# Autodesk Inventor assembly: Shield_100
(part 2 of 2)
- C:\Users\dvorakj\Documents\Inventor\Bakalarka\altium export\NUCLEO-F411RE_PCB_TOP_Designators_Varsay_X_8Dlan_416.ipt
- C:\Users\dvorakj\Documents\Inventor\Bakalarka\altium export\NUCLEO-F411RE_PCB_TOP_Designators_Varsay_X_8Dlan_417.ipt
- C:\Users\dvorakj\Documents\Inventor\Bakalarka\altium export\NUCLEO-F411RE_PCB_TOP_Designators_Varsay_X_8Dlan_418.ipt
- C:\Users\dvorakj\Documents\Inventor\Bakalarka\altium export\NUCLEO-F411RE_PCB_TOP_Designators_Varsay_X_8Dlan_419.ipt
- C:\Users\dvorakj\Documents\Inventor\Bakalarka\altium export\NUCLEO-F411RE_PCB_TOP_Designators_Varsay_X_8Dlan_420.ipt
- C:\Users\dvorakj\Documents\Inventor\Bakalarka\altium export\NUCLEO-F411RE_PCB_TOP_Designators_Varsay_X_8Dlan_421.ipt
- C:\Users\dvorakj\Documents\Inventor\Bakalarka\altium export\NUCLEO-F411RE_PCB_TOP_Designators_Varsay_X_8Dlan_422.ipt
- C:\Users\dvorakj\Documents\Inventor\Bakalarka\altium export\NUCLEO-F411RE_PCB_TOP_Designators_Varsay_X_8Dlan_423.ipt
- C:\Users\dvorakj\Documents\Inventor\Bakalarka\altium export\NUCLEO-F411RE_PCB_TOP_Designators_Varsay_X_8Dlan_424.ipt
- C:\Users\dvorakj\Documents\Inventor\Bakalarka\altium export\NUCLEO-F411RE_PCB_TOP_Designators_Varsay_X_8Dlan_425.ipt
- C:\Users\dvorakj\Documents\Inventor\Bakalarka\altium export\NUCLEO-F411RE_PCB_TOP_Designators_Varsay_X_8Dlan_426.ipt
- C:\Users\dvorakj\Documents\Inventor\Bakalarka\altium export\NUCLEO-F411RE_PCB_TOP_Designators_Varsay_X_8Dlan_427.ipt
- C:\Users\dvorakj\Documents\Inventor\Bakalarka\altium export\NUCLEO-F411RE_PCB_TOP_Designators_Varsay_X_8Dlan_428.ipt
- C:\Users\dvorakj\Documents\Inventor\Bakalarka\altium export\NUCLEO-F411RE_PCB_TOP_Designators_Varsay_X_8Dlan_429.ipt
- C:\Users\dvorakj\Documents\Inventor\Bakalarka\altium export\NUCLEO-F411RE_PCB_TOP_Designators_Varsay_X_8Dlan_430.ipt
- C:\Users\dvorakj\Documents\Inventor\Bakalarka\altium export\NUCLEO-F411RE_PCB_TOP_Designators_Varsay_X_8Dlan_431.ipt
- C:\Users\dvorakj\Documents\Inventor\Bakalarka\altium export\NUCLEO-F411RE_PCB_TOP_Designators_Varsay_X_8Dlan_432.ipt
- C:\Users\dvorakj\Documents\Inventor\Bakalarka\altium export\NUCLEO-F411RE_PCB_TOP_Designators_Varsay_X_8Dlan_433.ipt
- C:\Users\dvorakj\Documents\Inventor\Bakalarka\altium export\NUCLEO-F411RE_PCB_TOP_Designators_Varsay_X_8Dlan_434.ipt
- C:\Users\dvorakj\Documents\Inventor\Bakalarka\altium export\NUCLEO-F411RE_PCB_TOP_Designators_Varsay_X_8Dlan_435.ipt
- C:\Users\dvorakj\Documents\Inventor\Bakalarka\altium export\NUCLEO-F411RE_PCB_TOP_Designators_Varsay_X_8Dlan_436.ipt
- C:\Users\dvorakj\Documents\Inventor\Bakalarka\altium export\NUCLEO-F411RE_PCB_TOP_Designators_Varsay_X_8Dlan_437.ipt
- C:\Users\dvorakj\Documents\Inventor\Bakalarka\altium export\NUCLEO-F411RE_PCB_TOP_Designators_Varsay_X_8Dlan_438.ipt
- C:\Users\dvorakj\Documents\Inventor\Bakalarka\altium export\NUCLEO-F411RE_PCB_TOP_Designators_Varsay_X_8Dlan_439.ipt
- C:\Users\dvorakj\Documents\Inventor\Bakalarka\altium export\NUCLEO-F411RE_PCB_TOP_Designators_Varsay_X_8Dlan_440.ipt
- C:\Users\dvorakj\Documents\Inventor\Bakalarka\altium export\NUCLEO-F411RE_PCB_TOP_Designators_Varsay_X_8Dlan_441.ipt
- C:\Users\dvorakj\Documents\Inventor\Bakalarka\altium export\NUCLEO-F411RE_PCB_TOP_Designators_Varsay_X_8Dlan_442.ipt
- C:\Users\dvorakj\Documents\Inventor\Bakalarka\altium export\NUCLEO-F411RE_PCB_TOP_Designators_Varsay_X_8Dlan_443.ipt
- C:\Users\dvorakj\Documents\Inventor\Bakalarka\altium export\NUCLEO-F411RE_PCB_TOP_Designators_Varsay_X_8Dlan_444.ipt
- C:\Users\dvorakj\Documents\Inventor\Bakalarka\altium export\NUCLEO-F411RE_PCB_TOP_Designators_Varsay_X_8Dlan_445.ipt
- C:\Users\dvorakj\Documents\Inventor\Bakalarka\altium export\NUCLEO-F411RE_PCB_TOP_Designators_Varsay_X_8Dlan_446.ipt
- C:\Users\dvorakj\Documents\Inventor\Bakalarka\altium export\NUCLEO-F411RE_PCB_TOP_Designators_Varsay_X_8Dlan_447.ipt
- C:\Users\dvorakj\Documents\Inventor\Bakalarka\altium export\NUCLEO-F411RE_PCB_TOP_Designators_Varsay_X_8Dlan_448.ipt
- C:\Users\dvorakj\Documents\Inventor\Bakalarka\altium export\NUCLEO-F411RE_PCB_TOP_Designators_Varsay_X_8Dlan_449.ipt
- C:\Users\dvorakj\Documents\Inventor\Bakalarka\altium export\NUCLEO-F411RE_PCB_TOP_Designators_Varsay_X_8Dlan_450.ipt
- C:\Users\dvorakj\Documents\Inventor\Bakalarka\altium export\NUCLEO-F411RE_PCB_TOP_Designators_Varsay_X_8Dlan_451.ipt
- C:\Users\dvorakj\Documents\Inventor\Bakalarka\altium export\NUCLEO-F411RE_PCB_TOP_Designators_Varsay_X_8Dlan_452.ipt
- C:\Users\dvorakj\Documents\Inventor\Bakalarka\altium export\NUCLEO-F411RE_PCB_TOP_Designators_Varsay_X_8Dlan_453.ipt
- C:\Users\dvorakj\Documents\Inventor\Bakalarka\altium export\NUCLEO-F411RE_PCB_TOP_Designators_Varsay_X_8Dlan_454.ipt
- C:\Users\dvorakj\Documents\Inventor\Bakalarka\altium export\NUCLEO-F411RE_PCB_TOP_Designators_Varsay_X_8Dlan_455.ipt
- C:\Users\dvorakj\Documents\Inventor\Bakalarka\altium export\NUCLEO-F411RE_PCB_TOP_Designators_Varsay_X_8Dlan_456.ipt
- C:\Users\dvorakj\Documents\Inventor\Bakalarka\altium export\NUCLEO-F411RE_PCB_TOP_Designators_Varsay_X_8Dlan_457.ipt
- C:\Users\dvorakj\Documents\Inventor\Bakalarka\altium export\NUCLEO-F411RE_PCB_TOP_Designators_Varsay_X_8Dlan_458.ipt
- C:\Users\dvorakj\Documents\Inventor\Bakalarka\altium export\NUCLEO-F411RE_PCB_TOP_Designators_Varsay_X_8Dlan_459.ipt
- C:\Users\dvorakj\Documents\Inventor\Bakalarka\altium export\NUCLEO-F411RE_PCB_TOP_Designators_Varsay_X_8Dlan_460.ipt
- C:\Users\dvorakj\Documents\Inventor\Bakalarka\altium export\NUCLEO-F411RE_PCB_TOP_Designators_Varsay_X_8Dlan_461.ipt
- C:\Users\dvorakj\Documents\Inventor\Bakalarka\altium export\NUCLEO-F411RE_PCB_TOP_Designators_Varsay_X_8Dlan_462.ipt
- C:\Users\dvorakj\Documents\Inventor\Bakalarka\altium export\NUCLEO-F411RE_PCB_TOP_Designators_Varsay_X_8Dlan_463.ipt
- C:\Users\dvorakj\Documents\Inventor\Bakalarka\altium export\NUCLEO-F411RE_PCB_TOP_Designators_Varsay_X_8Dlan_464.ipt
- C:\Users\dvorakj\Documents\Inventor\Bakalarka\altium export\NUCLEO-F411RE_PCB_TOP_Designators_Varsay_X_8Dlan_465.ipt
- C:\Users\dvorakj\Documents\Inventor\Bakalarka\altium export\NUCLEO-F411RE_PCB_TOP_Designators_Varsay_X_8Dlan_466.ipt
- C:\Users\dvorakj\Documents\Inventor\Bakalarka\altium export\NUCLEO-F411RE_PCB_TOP_Designators_Varsay_X_8Dlan_467.ipt
- C:\Users\dvorakj\Documents\Inventor\Bakalarka\altium export\NUCLEO-F411RE_PCB_TOP_Designators_Varsay_X_8Dlan_468.ipt
- C:\Users\dvorakj\Documents\Inventor\Bakalarka\altium export\NUCLEO-F411RE_PCB_TOP_Designators_Varsay_X_8Dlan_469.ipt
- C:\Users\dvorakj\Documents\Inventor\Bakalarka\altium export\NUCLEO-F411RE_PCB_TOP_Designators_Varsay_X_8Dlan_470.ipt
- C:\Users\dvorakj\Documents\Inventor\Bakalarka\altium export\NUCLEO-F411RE_PCB_TOP_Designators_Varsay_X_8Dlan_471.ipt
- C:\Users\dvorakj\Documents\Inventor\Bakalarka\altium export\NUCLEO-F411RE_PCB_TOP_Designators_Varsay_X_8Dlan_472.ipt
- C:\Users\dvorakj\Documents\Inventor\Bakalarka\altium export\NUCLEO-F411RE_PCB_TOP_Designators_Varsay_X_8Dlan_473.ipt
- C:\Users\dvorakj\Documents\Inventor\Bakalarka\altium export\NUCLEO-F411RE_PCB_TOP_Designators_Varsay_X_8Dlan_474.ipt
- C:\Users\dvorakj\Documents\Inventor\Bakalarka\altium export\NUCLEO-F411RE_PCB_TOP_Designators_Varsay_X_8Dlan_475.ipt
- C:\Users\dvorakj\Documents\Inventor\Bakalarka\altium export\NUCLEO-F411RE_PCB_TOP_Designators_Varsay_X_8Dlan_476.ipt
- C:\Users\dvorakj\Documents\Inventor\Bakalarka\altium export\NUCLEO-F411RE_PCB_TOP_Designators_Varsay_X_8Dlan_477.ipt
- C:\Users\dvorakj\Documents\Inventor\Bakalarka\altium export\NUCLEO-F411RE_PCB_TOP_Designators_Varsay_X_8Dlan_478.ipt
- C:\Users\dvorakj\Documents\Inventor\Bakalarka\altium export\NUCLEO-F411RE_PCB_TOP_Designators_Varsay_X_8Dlan_479.ipt
- C:\Users\dvorakj\Documents\Inventor\Bakalarka\altium export\NUCLEO-F411RE_PCB_TOP_Designators_Varsay_X_8Dlan_480.ipt
- C:\Users\dvorakj\Documents\Inventor\Bakalarka\altium export\NUCLEO-F411RE_PCB_TOP_Designators_Varsay_X_8Dlan_481.ipt
- C:\Users\dvorakj\Documents\Inventor\Bakalarka\altium export\NUCLEO-F411RE_PCB_TOP_Designators_Varsay_X_8Dlan_482.ipt
- C:\Users\dvorakj\Documents\Inventor\Bakalarka\altium export\NUCLEO-F411RE_PCB_TOP_Designators_Varsay_X_8Dlan_483.ipt
- C:\Users\dvorakj\Documents\Inventor\Bakalarka\altium export\NUCLEO-F411RE_PCB_TOP_Designators_Varsay_X_8Dlan_484.ipt
- C:\Users\dvorakj\Documents\Inventor\Bakalarka\altium export\NUCLEO-F411RE_PCB_TOP_Designators_Varsay_X_8Dlan_485.ipt
- C:\Users\dvorakj\Documents\Inventor\Bakalarka\altium export\NUCLEO-F411RE_PCB_TOP_Designators_Varsay_X_8Dlan_486.ipt
- C:\Users\dvorakj\Documents\Inventor\Bakalarka\altium export\NUCLEO-F411RE_PCB_TOP_Designators_Varsay_X_8Dlan_487.ipt
- C:\Users\dvorakj\Documents\Inventor\Bakalarka\altium export\NUCLEO-F411RE_PCB_TOP_Designators_Varsay_X_8Dlan_488.ipt
- C:\Users\dvorakj\Documents\Inventor\Bakalarka\altium export\NUCLEO-F411RE_PCB_TOP_Designators_Varsay_X_8Dlan_489.ipt
- C:\Users\dvorakj\Documents\Inventor\Bakalarka\altium export\NUCLEO-F411RE_PCB_TOP_Designators_Varsay_X_8Dlan_490.ipt
- C:\Users\dvorakj\Documents\Inventor\Bakalarka\altium export\NUCLEO-F411RE_PCB_TOP_Designators_Varsay_X_8Dlan_491.ipt
- C:\Users\dvorakj\Documents\Inventor\Bakalarka\altium export\NUCLEO-F411RE_PCB_TOP_Designators_Varsay_X_8Dlan_492.ipt
- C:\Users\dvorakj\Documents\Inventor\Bakalarka\altium export\NUCLEO-F411RE_PCB_TOP_Designators_Varsay_X_8Dlan_493.ipt
- C:\Users\dvorakj\Documents\Inventor\Bakalarka\altium export\NUCLEO-F411RE_PCB_TOP_Designators_Varsay_X_8Dlan_494.ipt
- C:\Users\dvorakj\Documents\Inventor\Bakalarka\altium export\NUCLEO-F411RE_PCB_TOP_Designators_Varsay_X_8Dlan_495.ipt
- C:\Users\dvorakj\Documents\Inventor\Bakalarka\altium export\NUCLEO-F411RE_PCB_TOP_Designators_Varsay_X_8Dlan_496.ipt
- C:\Users\dvorakj\Documents\Inventor\Bakalarka\altium export\NUCLEO-F411RE_PCB_TOP_Designators_Varsay_X_8Dlan_497.ipt
- C:\Users\dvorakj\Documents\Inventor\Bakalarka\altium export\NUCLEO-F411RE_PCB_TOP_Designators_Varsay_X_8Dlan_498.ipt
- C:\Users\dvorakj\Documents\Inventor\Bakalarka\altium export\NUCLEO-F411RE_PCB_TOP_Designators_Varsay_X_8Dlan_499.ipt
- C:\Users\dvorakj\Documents\Inventor\Bakalarka\altium export\NUCLEO-F411RE_PCB_TOP_Designators_Varsay_X_8Dlan_500.ipt
- C:\Users\dvorakj\Documents\Inventor\Bakalarka\altium export\NUCLEO-F411RE_PCB_TOP_Designators_Varsay_X_8Dlan_501.ipt
- C:\Users\dvorakj\Documents\Inventor\Bakalarka\altium export\NUCLEO-F411RE_PCB_TOP_Designators_Varsay_X_8Dlan_502.ipt
- C:\Users\dvorakj\Documents\Inventor\Bakalarka\altium export\NUCLEO-F411RE_PCB_TOP_Designators_Varsay_X_8Dlan_503.ipt
- C:\Users\dvorakj\Documents\Inventor\Bakalarka\altium export\NUCLEO-F411RE_PCB_TOP_Designators_Varsay_X_8Dlan_504.ipt
- C:\Users\dvorakj\Documents\Inventor\Bakalarka\altium export\NUCLEO-F411RE_PCB_TOP_Designators_Varsay_X_8Dlan_505.ipt
- C:\Users\dvorakj\Documents\Inventor\Bakalarka\altium export\NUCLEO-F411RE_PCB_TOP_Designators_Varsay_X_8Dlan_506.ipt
- C:\Users\dvorakj\Documents\Inventor\Bakalarka\altium export\NUCLEO-F411RE_PCB_TOP_Designators_Varsay_X_8Dlan_507.ipt
- C:\Users\dvorakj\Documents\Inventor\Bakalarka\altium export\NUCLEO-F411RE_PCB_TOP_Designators_Varsay_X_8Dlan_508.ipt
- C:\Users\dvorakj\Documents\Inventor\Bakalarka\altium export\NUCLEO-F411RE_PCB_TOP_Designators_Varsay_X_8Dlan_509.ipt
- C:\Users\dvorakj\Documents\Inventor\Bakalarka\altium export\NUCLEO-F411RE_PCB_TOP_Designators_Varsay_X_8Dlan_510.ipt
- C:\Users\dvorakj\Documents\Inventor\Bakalarka\altium export\NUCLEO-F411RE_PCB_TOP_Designators_Varsay_X_8Dlan_511.ipt
- C:\Users\dvorakj\Documents\Inventor\Bakalarka\altium export\NUCLEO-F411RE_PCB_TOP_Designators_Varsay_X_8Dlan_512.ipt
- C:\Users\dvorakj\Documents\Inventor\Bakalarka\altium export\NUCLEO-F411RE_PCB_TOP_Designators_Varsay_X_8Dlan_513.ipt
- C:\Users\dvorakj\Documents\Inventor\Bakalarka\altium export\NUCLEO-F411RE_PCB_TOP_Designators_Varsay_X_8Dlan_514.ipt
- C:\Users\dvorakj\Documents\Inventor\Bakalarka\altium export\NUCLEO-F411RE_PCB_TOP_Designators_Varsay_X_8Dlan_515.ipt
- C:\Users\dvorakj\Documents\Inventor\Bakalarka\altium export\NUCLEO-F411RE_PCB_TOP_Designators_Varsay_X_8Dlan_516.ipt
- C:\Users\dvorakj\Documents\Inventor\Bakalarka\altium export\NUCLEO-F411RE_PCB_TOP_Designators_Varsay_X_8Dlan_517.ipt
- C:\Users\dvorakj\Documents\Inventor\Bakalarka\altium export\NUCLEO-F411RE_PCB_TOP_Designators_Varsay_X_8Dlan_518.ipt
- C:\Users\dvorakj\Documents\Inventor\Bakalarka\altium export\NUCLEO-F411RE_PCB_TOP_Designators_Varsay_X_8Dlan_519.ipt
- C:\Users\dvorakj\Documents\Inventor\Bakalarka\altium export\NUCLEO-F411RE_PCB_TOP_Designators_Varsay_X_8Dlan_520.ipt
- C:\Users\dvorakj\Documents\Inventor\Bakalarka\altium export\NUCLEO-F411RE_PCB_TOP_Designators_Varsay_X_8Dlan_521.ipt
- C:\Users\dvorakj\Documents\Inventor\Bakalarka\altium export\NUCLEO-F411RE_PCB_TOP_Designators_Varsay_X_8Dlan_522.ipt
- C:\Users\dvorakj\Documents\Inventor\Bakalarka\altium export\NUCLEO-F411RE_PCB_TOP_Designators_Varsay_X_8Dlan_523.ipt
- C:\Users\dvorakj\Documents\Inventor\Bakalarka\altium export\NUCLEO-F411RE_PCB_TOP_Designators_Varsay_X_8Dlan_524.ipt
- C:\Users\dvorakj\Documents\Inventor\Bakalarka\altium export\NUCLEO-F411RE_PCB_TOP_Designators_Varsay_X_8Dlan_525.ipt
- C:\Users\dvorakj\Documents\Inventor\Bakalarka\altium export\NUCLEO-F411RE_PCB_TOP_Designators_Varsay_X_8Dlan_526.ipt
- C:\Users\dvorakj\Documents\Inventor\Bakalarka\altium export\NUCLEO-F411RE_PCB_TOP_Designators_Varsay_X_8Dlan_527.ipt
- C:\Users\dvorakj\Documents\Inventor\Bakalarka\altium export\NUCLEO-F411RE_PCB_TOP_Designators_Varsay_X_8Dlan_528.ipt
- C:\Users\dvorakj\Documents\Inventor\Bakalarka\altium export\NUCLEO-F411RE_PCB_TOP_Designators_Varsay_X_8Dlan_529.ipt
- C:\Users\dvorakj\Documents\Inventor\Bakalarka\altium export\NUCLEO-F411RE_PCB_TOP_Designators_Varsay_X_8Dlan_530.ipt
- C:\Users\dvorakj\Documents\Inventor\Bakalarka\altium export\NUCLEO-F411RE_PCB_TOP_Designators_Varsay_X_8Dlan_531.ipt
## Components (532 placed, 532 different names)
1. NUCLEO-F411RE_PCB_TOP_Designators_Varsay_X_8Dlan
2. NUCLEO-F411RE_PCB_TOP_Designators_Varsay_X_8Dlan_1
3. NUCLEO-F411RE_PCB_TOP_Designators_Varsay_X_8Dlan_2
4. NUCLEO-F411RE_PCB_TOP_Designators_Varsay_X_8Dlan_3
5. NUCLEO-F411RE_PCB_TOP_Designators_Varsay_X_8Dlan_4
6. NUCLEO-F411RE_PCB_TOP_Designators_Varsay_X_8Dlan_5
7. NUCLEO-F411RE_PCB_TOP_Designators_Varsay_X_8Dlan_6
8. NUCLEO-F411RE_PCB_TOP_Designators_Varsay_X_8Dlan_7
9. NUCLEO-F411RE_PCB_TOP_Designators_Varsay_X_8Dlan_8
10. NUCLEO-F411RE_PCB_TOP_Designators_Varsay_X_8Dlan_9
11. NUCLEO-F411RE_PCB_TOP_Designators_Varsay_X_8Dlan_10
12. NUCLEO-F411RE_PCB_TOP_Designators_Varsay_X_8Dlan_11
13. NUCLEO-F411RE_PCB_TOP_Designators_Varsay_X_8Dlan_12
14. NUCLEO-F411RE_PCB_TOP_Designators_Varsay_X_8Dlan_13
15. NUCLEO-F411RE_PCB_TOP_Designators_Varsay_X_8Dlan_14
16. NUCLEO-F411RE_PCB_TOP_Designators_Varsay_X_8Dlan_15
17. NUCLEO-F411RE_PCB_TOP_Designators_Varsay_X_8Dlan_16
18. NUCLEO-F411RE_PCB_TOP_Designators_Varsay_X_8Dlan_17
19. NUCLEO-F411RE_PCB_TOP_Designators_Varsay_X_8Dlan_18
20. NUCLEO-F411RE_PCB_TOP_Designators_Varsay_X_8Dlan_19
21. NUCLEO-F411RE_PCB_TOP_Designators_Varsay_X_8Dlan_20
22. NUCLEO-F411RE_PCB_TOP_Designators_Varsay_X_8Dlan_21
23. NUCLEO-F411RE_PCB_TOP_Designators_Varsay_X_8Dlan_22
24. NUCLEO-F411RE_PCB_TOP_Designators_Varsay_X_8Dlan_23
25. NUCLEO-F411RE_PCB_TOP_Designators_Varsay_X_8Dlan_24
26. NUCLEO-F411RE_PCB_TOP_Designators_Varsay_X_8Dlan_25
27. NUCLEO-F411RE_PCB_TOP_Designators_Varsay_X_8Dlan_26
28. NUCLEO-F411RE_PCB_TOP_Designators_Varsay_X_8Dlan_27
29. NUCLEO-F411RE_PCB_TOP_Designators_Varsay_X_8Dlan_28
30. NUCLEO-F411RE_PCB_TOP_Designators_Varsay_X_8Dlan_29
31. NUCLEO-F411RE_PCB_TOP_Designators_Varsay_X_8Dlan_30
32. NUCLEO-F411RE_PCB_TOP_Designators_Varsay_X_8Dlan_31
33. NUCLEO-F411RE_PCB_TOP_Designators_Varsay_X_8Dlan_32
34. NUCLEO-F411RE_PCB_TOP_Designators_Varsay_X_8Dlan_33
35. NUCLEO-F411RE_PCB_TOP_Designators_Varsay_X_8Dlan_34
36. NUCLEO-F411RE_PCB_TOP_Designators_Varsay_X_8Dlan_35
37. NUCLEO-F411RE_PCB_TOP_Designators_Varsay_X_8Dlan_36
38. NUCLEO-F411RE_PCB_TOP_Designators_Varsay_X_8Dlan_37
39. NUCLEO-F411RE_PCB_TOP_Designators_Varsay_X_8Dlan_38
40. NUCLEO-F411RE_PCB_TOP_Designators_Varsay_X_8Dlan_39
41. NUCLEO-F411RE_PCB_TOP_Designators_Varsay_X_8Dlan_40
42. NUCLEO-F411RE_PCB_TOP_Designators_Varsay_X_8Dlan_41
43. NUCLEO-F411RE_PCB_TOP_Designators_Varsay_X_8Dlan_42
44. NUCLEO-F411RE_PCB_TOP_Designators_Varsay_X_8Dlan_43
45. NUCLEO-F411RE_PCB_TOP_Designators_Varsay_X_8Dlan_44
46. NUCLEO-F411RE_PCB_TOP_Designators_Varsay_X_8Dlan_45
47. NUCLEO-F411RE_PCB_TOP_Designators_Varsay_X_8Dlan_46
48. NUCLEO-F411RE_PCB_TOP_Designators_Varsay_X_8Dlan_47
49. NUCLEO-F411RE_PCB_TOP_Designators_Varsay_X_8Dlan_48
50. NUCLEO-F411RE_PCB_TOP_Designators_Varsay_X_8Dlan_49
51. NUCLEO-F411RE_PCB_TOP_Designators_Varsay_X_8Dlan_50
52. NUCLEO-F411RE_PCB_TOP_Designators_Varsay_X_8Dlan_51
53. NUCLEO-F411RE_PCB_TOP_Designators_Varsay_X_8Dlan_52
54. NUCLEO-F411RE_PCB_TOP_Designators_Varsay_X_8Dlan_53
55. NUCLEO-F411RE_PCB_TOP_Designators_Varsay_X_8Dlan_54
56. NUCLEO-F411RE_PCB_TOP_Designators_Varsay_X_8Dlan_55
57. NUCLEO-F411RE_PCB_TOP_Designators_Varsay_X_8Dlan_56
58. NUCLEO-F411RE_PCB_TOP_Designators_Varsay_X_8Dlan_57
59. NUCLEO-F411RE_PCB_TOP_Designators_Varsay_X_8Dlan_58
60. NUCLEO-F411RE_PCB_TOP_Designators_Varsay_X_8Dlan_59
61. NUCLEO-F411RE_PCB_TOP_Designators_Varsay_X_8Dlan_60
62. NUCLEO-F411RE_PCB_TOP_Designators_Varsay_X_8Dlan_61
63. NUCLEO-F411RE_PCB_TOP_Designators_Varsay_X_8Dlan_62
64. NUCLEO-F411RE_PCB_TOP_Designators_Varsay_X_8Dlan_63
65. NUCLEO-F411RE_PCB_TOP_Designators_Varsay_X_8Dlan_64
66. NUCLEO-F411RE_PCB_TOP_Designators_Varsay_X_8Dlan_65
67. NUCLEO-F411RE_PCB_TOP_Designators_Varsay_X_8Dlan_66
68. NUCLEO-F411RE_PCB_TOP_Designators_Varsay_X_8Dlan_67
69. NUCLEO-F411RE_PCB_TOP_Designators_Varsay_X_8Dlan_68
70. NUCLEO-F411RE_PCB_TOP_Designators_Varsay_X_8Dlan_69
71. NUCLEO-F411RE_PCB_TOP_Designators_Varsay_X_8Dlan_70
72. NUCLEO-F411RE_PCB_TOP_Designators_Varsay_X_8Dlan_71
73. NUCLEO-F411RE_PCB_TOP_Designators_Varsay_X_8Dlan_72
74. NUCLEO-F411RE_PCB_TOP_Designators_Varsay_X_8Dlan_73
75. NUCLEO-F411RE_PCB_TOP_Designators_Varsay_X_8Dlan_74
76. NUCLEO-F411RE_PCB_TOP_Designators_Varsay_X_8Dlan_75
77. NUCLEO-F411RE_PCB_TOP_Designators_Varsay_X_8Dlan_76
78. NUCLEO-F411RE_PCB_TOP_Designators_Varsay_X_8Dlan_77
79. NUCLEO-F411RE_PCB_TOP_Designators_Varsay_X_8Dlan_78
80. NUCLEO-F411RE_PCB_TOP_Designators_Varsay_X_8Dlan_79
81. NUCLEO-F411RE_PCB_TOP_Designators_Varsay_X_8Dlan_80
82. NUCLEO-F411RE_PCB_TOP_Designators_Varsay_X_8Dlan_81
83. NUCLEO-F411RE_PCB_TOP_Designators_Varsay_X_8Dlan_82
84. NUCLEO-F411RE_PCB_TOP_Designators_Varsay_X_8Dlan_83
85. NUCLEO-F411RE_PCB_TOP_Designators_Varsay_X_8Dlan_84
86. NUCLEO-F411RE_PCB_TOP_Designators_Varsay_X_8Dlan_85
87. NUCLEO-F411RE_PCB_TOP_Designators_Varsay_X_8Dlan_86
88. NUCLEO-F411RE_PCB_TOP_Designators_Varsay_X_8Dlan_87
89. NUCLEO-F411RE_PCB_TOP_Designators_Varsay_X_8Dlan_88
90. NUCLEO-F411RE_PCB_TOP_Designators_Varsay_X_8Dlan_89
91. NUCLEO-F411RE_PCB_TOP_Designators_Varsay_X_8Dlan_90
92. NUCLEO-F411RE_PCB_TOP_Designators_Varsay_X_8Dlan_91
93. NUCLEO-F411RE_PCB_TOP_Designators_Varsay_X_8Dlan_92
94. NUCLEO-F411RE_PCB_TOP_Designators_Varsay_X_8Dlan_93
95. NUCLEO-F411RE_PCB_TOP_Designators_Varsay_X_8Dlan_94
96. NUCLEO-F411RE_PCB_TOP_Designators_Varsay_X_8Dlan_95
97. NUCLEO-F411RE_PCB_TOP_Designators_Varsay_X_8Dlan_96
98. NUCLEO-F411RE_PCB_TOP_Designators_Varsay_X_8Dlan_97
99. NUCLEO-F411RE_PCB_TOP_Designators_Varsay_X_8Dlan_98
100. NUCLEO-F411RE_PCB_TOP_Designators_Varsay_X_8Dlan_99
101. NUCLEO-F411RE_PCB_TOP_Designators_Varsay_X_8Dlan_100
102. NUCLEO-F411RE_PCB_TOP_Designators_Varsay_X_8Dlan_101
103. NUCLEO-F411RE_PCB_TOP_Designators_Varsay_X_8Dlan_102
104. NUCLEO-F411RE_PCB_TOP_Designators_Varsay_X_8Dlan_103
105. NUCLEO-F411RE_PCB_TOP_Designators_Varsay_X_8Dlan_104
106. NUCLEO-F411RE_PCB_TOP_Designators_Varsay_X_8Dlan_105
107. NUCLEO-F411RE_PCB_TOP_Designators_Varsay_X_8Dlan_106
108. NUCLEO-F411RE_PCB_TOP_Designators_Varsay_X_8Dlan_107
109. NUCLEO-F411RE_PCB_TOP_Designators_Varsay_X_8Dlan_108
110. NUCLEO-F411RE_PCB_TOP_Designators_Varsay_X_8Dlan_109
111. NUCLEO-F411RE_PCB_TOP_Designators_Varsay_X_8Dlan_110
112. NUCLEO-F411RE_PCB_TOP_Designators_Varsay_X_8Dlan_111
113. NUCLEO-F411RE_PCB_TOP_Designators_Varsay_X_8Dlan_112
114. NUCLEO-F411RE_PCB_TOP_Designators_Varsay_X_8Dlan_113
115. NUCLEO-F411RE_PCB_TOP_Designators_Varsay_X_8Dlan_114
116. NUCLEO-F411RE_PCB_TOP_Designators_Varsay_X_8Dlan_115
117. NUCLEO-F411RE_PCB_TOP_Designators_Varsay_X_8Dlan_116
118. NUCLEO-F411RE_PCB_TOP_Designators_Varsay_X_8Dlan_117
119. NUCLEO-F411RE_PCB_TOP_Designators_Varsay_X_8Dlan_118
120. NUCLEO-F411RE_PCB_TOP_Designators_Varsay_X_8Dlan_119
121. NUCLEO-F411RE_PCB_TOP_Designators_Varsay_X_8Dlan_120
122. NUCLEO-F411RE_PCB_TOP_Designators_Varsay_X_8Dlan_121
123. NUCLEO-F411RE_PCB_TOP_Designators_Varsay_X_8Dlan_122
124. NUCLEO-F411RE_PCB_TOP_Designators_Varsay_X_8Dlan_123
125. NUCLEO-F411RE_PCB_TOP_Designators_Varsay_X_8Dlan_124
126. NUCLEO-F411RE_PCB_TOP_Designators_Varsay_X_8Dlan_125
127. NUCLEO-F411RE_PCB_TOP_Designators_Varsay_X_8Dlan_126
128. NUCLEO-F411RE_PCB_TOP_Designators_Varsay_X_8Dlan_127
129. NUCLEO-F411RE_PCB_TOP_Designators_Varsay_X_8Dlan_128
130. NUCLEO-F411RE_PCB_TOP_Designators_Varsay_X_8Dlan_129
131. NUCLEO-F411RE_PCB_TOP_Designators_Varsay_X_8Dlan_130
132. NUCLEO-F411RE_PCB_TOP_Designators_Varsay_X_8Dlan_131
133. NUCLEO-F411RE_PCB_TOP_Designators_Varsay_X_8Dlan_132
134. NUCLEO-F411RE_PCB_TOP_Designators_Varsay_X_8Dlan_133
135. NUCLEO-F411RE_PCB_TOP_Designators_Varsay_X_8Dlan_134
136. NUCLEO-F411RE_PCB_TOP_Designators_Varsay_X_8Dlan_135
137. NUCLEO-F411RE_PCB_TOP_Designators_Varsay_X_8Dlan_136
138. NUCLEO-F411RE_PCB_TOP_Designators_Varsay_X_8Dlan_137
139. NUCLEO-F411RE_PCB_TOP_Designators_Varsay_X_8Dlan_138
140. NUCLEO-F411RE_PCB_TOP_Designators_Varsay_X_8Dlan_139
141. NUCLEO-F411RE_PCB_TOP_Designators_Varsay_X_8Dlan_140
142. NUCLEO-F411RE_PCB_TOP_Designators_Varsay_X_8Dlan_141
143. NUCLEO-F411RE_PCB_TOP_Designators_Varsay_X_8Dlan_142
144. NUCLEO-F411RE_PCB_TOP_Designators_Varsay_X_8Dlan_143
145. NUCLEO-F411RE_PCB_TOP_Designators_Varsay_X_8Dlan_144
146. NUCLEO-F411RE_PCB_TOP_Designators_Varsay_X_8Dlan_145
147. NUCLEO-F411RE_PCB_TOP_Designators_Varsay_X_8Dlan_146
148. NUCLEO-F411RE_PCB_TOP_Designators_Varsay_X_8Dlan_147
149. NUCLEO-F411RE_PCB_TOP_Designators_Varsay_X_8Dlan_148
150. NUCLEO-F411RE_PCB_TOP_Designators_Varsay_X_8Dlan_149
151. NUCLEO-F411RE_PCB_TOP_Designators_Varsay_X_8Dlan_150
152. NUCLEO-F411RE_PCB_TOP_Designators_Varsay_X_8Dlan_151
153. NUCLEO-F411RE_PCB_TOP_Designators_Varsay_X_8Dlan_152
154. NUCLEO-F411RE_PCB_TOP_Designators_Varsay_X_8Dlan_153
155. NUCLEO-F411RE_PCB_TOP_Designators_Varsay_X_8Dlan_154
156. NUCLEO-F411RE_PCB_TOP_Designators_Varsay_X_8Dlan_155
157. NUCLEO-F411RE_PCB_TOP_Designators_Varsay_X_8Dlan_156
158. NUCLEO-F411RE_PCB_TOP_Designators_Varsay_X_8Dlan_157
159. NUCLEO-F411RE_PCB_TOP_Designators_Varsay_X_8Dlan_158
160. NUCLEO-F411RE_PCB_TOP_Designators_Varsay_X_8Dlan_159
161. NUCLEO-F411RE_PCB_TOP_Designators_Varsay_X_8Dlan_160
162. NUCLEO-F411RE_PCB_TOP_Designators_Varsay_X_8Dlan_161
163. NUCLEO-F411RE_PCB_TOP_Designators_Varsay_X_8Dlan_162
164. NUCLEO-F411RE_PCB_TOP_Designators_Varsay_X_8Dlan_163
165. NUCLEO-F411RE_PCB_TOP_Designators_Varsay_X_8Dlan_164
166. NUCLEO-F411RE_PCB_TOP_Designators_Varsay_X_8Dlan_165
167. NUCLEO-F411RE_PCB_TOP_Designators_Varsay_X_8Dlan_166
168. NUCLEO-F411RE_PCB_TOP_Designators_Varsay_X_8Dlan_167
169. NUCLEO-F411RE_PCB_TOP_Designators_Varsay_X_8Dlan_168
170. NUCLEO-F411RE_PCB_TOP_Designators_Varsay_X_8Dlan_169
171. NUCLEO-F411RE_PCB_TOP_Designators_Varsay_X_8Dlan_170
172. NUCLEO-F411RE_PCB_TOP_Designators_Varsay_X_8Dlan_171
173. NUCLEO-F411RE_PCB_TOP_Designators_Varsay_X_8Dlan_172
174. NUCLEO-F411RE_PCB_TOP_Designators_Varsay_X_8Dlan_173
175. NUCLEO-F411RE_PCB_TOP_Designators_Varsay_X_8Dlan_174
176. NUCLEO-F411RE_PCB_TOP_Designators_Varsay_X_8Dlan_175
177. NUCLEO-F411RE_PCB_TOP_Designators_Varsay_X_8Dlan_176
178. NUCLEO-F411RE_PCB_TOP_Designators_Varsay_X_8Dlan_177
179. NUCLEO-F411RE_PCB_TOP_Designators_Varsay_X_8Dlan_178
180. NUCLEO-F411RE_PCB_TOP_Designators_Varsay_X_8Dlan_179
181. NUCLEO-F411RE_PCB_TOP_Designators_Varsay_X_8Dlan_180
182. NUCLEO-F411RE_PCB_TOP_Designators_Varsay_X_8Dlan_181
183. NUCLEO-F411RE_PCB_TOP_Designators_Varsay_X_8Dlan_182
184. NUCLEO-F411RE_PCB_TOP_Designators_Varsay_X_8Dlan_183
185. NUCLEO-F411RE_PCB_TOP_Designators_Varsay_X_8Dlan_184
186. NUCLEO-F411RE_PCB_TOP_Designators_Varsay_X_8Dlan_185
187. NUCLEO-F411RE_PCB_TOP_Designators_Varsay_X_8Dlan_186
188. NUCLEO-F411RE_PCB_TOP_Designators_Varsay_X_8Dlan_187
189. NUCLEO-F411RE_PCB_TOP_Designators_Varsay_X_8Dlan_188
190. NUCLEO-F411RE_PCB_TOP_Designators_Varsay_X_8Dlan_189
191. NUCLEO-F411RE_PCB_TOP_Designators_Varsay_X_8Dlan_190
192. NUCLEO-F411RE_PCB_TOP_Designators_Varsay_X_8Dlan_191
193. NUCLEO-F411RE_PCB_TOP_Designators_Varsay_X_8Dlan_192
194. NUCLEO-F411RE_PCB_TOP_Designators_Varsay_X_8Dlan_193
195. NUCLEO-F411RE_PCB_TOP_Designators_Varsay_X_8Dlan_194
196. NUCLEO-F411RE_PCB_TOP_Designators_Varsay_X_8Dlan_195
197. NUCLEO-F411RE_PCB_TOP_Designators_Varsay_X_8Dlan_196
198. NUCLEO-F411RE_PCB_TOP_Designators_Varsay_X_8Dlan_197
199. NUCLEO-F411RE_PCB_TOP_Designators_Varsay_X_8Dlan_198
200. NUCLEO-F411RE_PCB_TOP_Designators_Varsay_X_8Dlan_199
201. NUCLEO-F411RE_PCB_TOP_Designators_Varsay_X_8Dlan_200
202. NUCLEO-F411RE_PCB_TOP_Designators_Varsay_X_8Dlan_201
203. NUCLEO-F411RE_PCB_TOP_Designators_Varsay_X_8Dlan_202
204. NUCLEO-F411RE_PCB_TOP_Designators_Varsay_X_8Dlan_203
205. NUCLEO-F411RE_PCB_TOP_Designators_Varsay_X_8Dlan_204
206. NUCLEO-F411RE_PCB_TOP_Designators_Varsay_X_8Dlan_205
207. NUCLEO-F411RE_PCB_TOP_Designators_Varsay_X_8Dlan_206
208. NUCLEO-F411RE_PCB_TOP_Designators_Varsay_X_8Dlan_207
209. NUCLEO-F411RE_PCB_TOP_Designators_Varsay_X_8Dlan_208
210. NUCLEO-F411RE_PCB_TOP_Designators_Varsay_X_8Dlan_209
211. NUCLEO-F411RE_PCB_TOP_Designators_Varsay_X_8Dlan_210
212. NUCLEO-F411RE_PCB_TOP_Designators_Varsay_X_8Dlan_211
213. NUCLEO-F411RE_PCB_TOP_Designators_Varsay_X_8Dlan_212
214. NUCLEO-F411RE_PCB_TOP_Designators_Varsay_X_8Dlan_213
215. NUCLEO-F411RE_PCB_TOP_Designators_Varsay_X_8Dlan_214
216. NUCLEO-F411RE_PCB_TOP_Designators_Varsay_X_8Dlan_215
217. NUCLEO-F411RE_PCB_TOP_Designators_Varsay_X_8Dlan_216
218. NUCLEO-F411RE_PCB_TOP_Designators_Varsay_X_8Dlan_217
219. NUCLEO-F411RE_PCB_TOP_Designators_Varsay_X_8Dlan_218
220. NUCLEO-F411RE_PCB_TOP_Designators_Varsay_X_8Dlan_219
221. NUCLEO-F411RE_PCB_TOP_Designators_Varsay_X_8Dlan_220
222. NUCLEO-F411RE_PCB_TOP_Designators_Varsay_X_8Dlan_221
223. NUCLEO-F411RE_PCB_TOP_Designators_Varsay_X_8Dlan_222
224. NUCLEO-F411RE_PCB_TOP_Designators_Varsay_X_8Dlan_223
225. NUCLEO-F411RE_PCB_TOP_Designators_Varsay_X_8Dlan_224
226. NUCLEO-F411RE_PCB_TOP_Designators_Varsay_X_8Dlan_225
227. NUCLEO-F411RE_PCB_TOP_Designators_Varsay_X_8Dlan_226
228. NUCLEO-F411RE_PCB_TOP_Designators_Varsay_X_8Dlan_227
229. NUCLEO-F411RE_PCB_TOP_Designators_Varsay_X_8Dlan_228
230. NUCLEO-F411RE_PCB_TOP_Designators_Varsay_X_8Dlan_229
231. NUCLEO-F411RE_PCB_TOP_Designators_Varsay_X_8Dlan_230
232. NUCLEO-F411RE_PCB_TOP_Designators_Varsay_X_8Dlan_231
233. NUCLEO-F411RE_PCB_TOP_Designators_Varsay_X_8Dlan_232
234. NUCLEO-F411RE_PCB_TOP_Designators_Varsay_X_8Dlan_233
235. NUCLEO-F411RE_PCB_TOP_Designators_Varsay_X_8Dlan_234
236. NUCLEO-F411RE_PCB_TOP_Designators_Varsay_X_8Dlan_235
237. NUCLEO-F411RE_PCB_TOP_Designators_Varsay_X_8Dlan_236
238. NUCLEO-F411RE_PCB_TOP_Designators_Varsay_X_8Dlan_237
239. NUCLEO-F411RE_PCB_TOP_Designators_Varsay_X_8Dlan_238
240. NUCLEO-F411RE_PCB_TOP_Designators_Varsay_X_8Dlan_239
241. NUCLEO-F411RE_PCB_TOP_Designators_Varsay_X_8Dlan_240
242. NUCLEO-F411RE_PCB_TOP_Designators_Varsay_X_8Dlan_241
243. NUCLEO-F411RE_PCB_TOP_Designators_Varsay_X_8Dlan_242
244. NUCLEO-F411RE_PCB_TOP_Designators_Varsay_X_8Dlan_243
245. NUCLEO-F411RE_PCB_TOP_Designators_Varsay_X_8Dlan_244
246. NUCLEO-F411RE_PCB_TOP_Designators_Varsay_X_8Dlan_245
247. NUCLEO-F411RE_PCB_TOP_Designators_Varsay_X_8Dlan_246
248. NUCLEO-F411RE_PCB_TOP_Designators_Varsay_X_8Dlan_247
249. NUCLEO-F411RE_PCB_TOP_Designators_Varsay_X_8Dlan_248
250. NUCLEO-F411RE_PCB_TOP_Designators_Varsay_X_8Dlan_249
251. NUCLEO-F411RE_PCB_TOP_Designators_Varsay_X_8Dlan_250
252. NUCLEO-F411RE_PCB_TOP_Designators_Varsay_X_8Dlan_251
253. NUCLEO-F411RE_PCB_TOP_Designators_Varsay_X_8Dlan_252
254. NUCLEO-F411RE_PCB_TOP_Designators_Varsay_X_8Dlan_253
255. NUCLEO-F411RE_PCB_TOP_Designators_Varsay_X_8Dlan_254
256. NUCLEO-F411RE_PCB_TOP_Designators_Varsay_X_8Dlan_255
257. NUCLEO-F411RE_PCB_TOP_Designators_Varsay_X_8Dlan_256
258. NUCLEO-F411RE_PCB_TOP_Designators_Varsay_X_8Dlan_257
259. NUCLEO-F411RE_PCB_TOP_Designators_Varsay_X_8Dlan_258
260. NUCLEO-F411RE_PCB_TOP_Designators_Varsay_X_8Dlan_259
261. NUCLEO-F411RE_PCB_TOP_Designators_Varsay_X_8Dlan_260
262. NUCLEO-F411RE_PCB_TOP_Designators_Varsay_X_8Dlan_261
263. NUCLEO-F411RE_PCB_TOP_Designators_Varsay_X_8Dlan_262
264. NUCLEO-F411RE_PCB_TOP_Designators_Varsay_X_8Dlan_263
265. NUCLEO-F411RE_PCB_TOP_Designators_Varsay_X_8Dlan_264
266. NUCLEO-F411RE_PCB_TOP_Designators_Varsay_X_8Dlan_265
267. NUCLEO-F411RE_PCB_TOP_Designators_Varsay_X_8Dlan_266
268. NUCLEO-F411RE_PCB_TOP_Designators_Varsay_X_8Dlan_267
269. NUCLEO-F411RE_PCB_TOP_Designators_Varsay_X_8Dlan_268
270. NUCLEO-F411RE_PCB_TOP_Designators_Varsay_X_8Dlan_269
271. NUCLEO-F411RE_PCB_TOP_Designators_Varsay_X_8Dlan_270
272. NUCLEO-F411RE_PCB_TOP_Designators_Varsay_X_8Dlan_271
273. NUCLEO-F411RE_PCB_TOP_Designators_Varsay_X_8Dlan_272
274. NUCLEO-F411RE_PCB_TOP_Designators_Varsay_X_8Dlan_273
275. NUCLEO-F411RE_PCB_TOP_Designators_Varsay_X_8Dlan_274
276. NUCLEO-F411RE_PCB_TOP_Designators_Varsay_X_8Dlan_275
277. NUCLEO-F411RE_PCB_TOP_Designators_Varsay_X_8Dlan_276
278. NUCLEO-F411RE_PCB_TOP_Designators_Varsay_X_8Dlan_277
279. NUCLEO-F411RE_PCB_TOP_Designators_Varsay_X_8Dlan_278
280. NUCLEO-F411RE_PCB_TOP_Designators_Varsay_X_8Dlan_279
281. NUCLEO-F411RE_PCB_TOP_Designators_Varsay_X_8Dlan_280
282. NUCLEO-F411RE_PCB_TOP_Designators_Varsay_X_8Dlan_281
283. NUCLEO-F411RE_PCB_TOP_Designators_Varsay_X_8Dlan_282
284. NUCLEO-F411RE_PCB_TOP_Designators_Varsay_X_8Dlan_283
285. NUCLEO-F411RE_PCB_TOP_Designators_Varsay_X_8Dlan_284
286. NUCLEO-F411RE_PCB_TOP_Designators_Varsay_X_8Dlan_285
287. NUCLEO-F411RE_PCB_TOP_Designators_Varsay_X_8Dlan_286
288. NUCLEO-F411RE_PCB_TOP_Designators_Varsay_X_8Dlan_287
289. NUCLEO-F411RE_PCB_TOP_Designators_Varsay_X_8Dlan_288
290. NUCLEO-F411RE_PCB_TOP_Designators_Varsay_X_8Dlan_289
291. NUCLEO-F411RE_PCB_TOP_Designators_Varsay_X_8Dlan_290
292. NUCLEO-F411RE_PCB_TOP_Designators_Varsay_X_8Dlan_291
293. NUCLEO-F411RE_PCB_TOP_Designators_Varsay_X_8Dlan_292
294. NUCLEO-F411RE_PCB_TOP_Designators_Varsay_X_8Dlan_293
295. NUCLEO-F411RE_PCB_TOP_Designators_Varsay_X_8Dlan_294
296. NUCLEO-F411RE_PCB_TOP_Designators_Varsay_X_8Dlan_295
297. NUCLEO-F411RE_PCB_TOP_Designators_Varsay_X_8Dlan_296
298. NUCLEO-F411RE_PCB_TOP_Designators_Varsay_X_8Dlan_297
299. NUCLEO-F411RE_PCB_TOP_Designators_Varsay_X_8Dlan_298
300. NUCLEO-F411RE_PCB_TOP_Designators_Varsay_X_8Dlan_299
301. NUCLEO-F411RE_PCB_TOP_Designators_Varsay_X_8Dlan_300
302. NUCLEO-F411RE_PCB_TOP_Designators_Varsay_X_8Dlan_301
303. NUCLEO-F411RE_PCB_TOP_Designators_Varsay_X_8Dlan_302
304. NUCLEO-F411RE_PCB_TOP_Designators_Varsay_X_8Dlan_303
305. NUCLEO-F411RE_PCB_TOP_Designators_Varsay_X_8Dlan_304
306. NUCLEO-F411RE_PCB_TOP_Designators_Varsay_X_8Dlan_305
307. NUCLEO-F411RE_PCB_TOP_Designators_Varsay_X_8Dlan_306
308. NUCLEO-F411RE_PCB_TOP_Designators_Varsay_X_8Dlan_307
309. NUCLEO-F411RE_PCB_TOP_Designators_Varsay_X_8Dlan_308
310. NUCLEO-F411RE_PCB_TOP_Designators_Varsay_X_8Dlan_309
311. NUCLEO-F411RE_PCB_TOP_Designators_Varsay_X_8Dlan_310
312. NUCLEO-F411RE_PCB_TOP_Designators_Varsay_X_8Dlan_311
313. NUCLEO-F411RE_PCB_TOP_Designators_Varsay_X_8Dlan_312
314. NUCLEO-F411RE_PCB_TOP_Designators_Varsay_X_8Dlan_313
315. NUCLEO-F411RE_PCB_TOP_Designators_Varsay_X_8Dlan_314
316. NUCLEO-F411RE_PCB_TOP_Designators_Varsay_X_8Dlan_315
317. NUCLEO-F411RE_PCB_TOP_Designators_Varsay_X_8Dlan_316
318. NUCLEO-F411RE_PCB_TOP_Designators_Varsay_X_8Dlan_317
319. NUCLEO-F411RE_PCB_TOP_Designators_Varsay_X_8Dlan_318
320. NUCLEO-F411RE_PCB_TOP_Designators_Varsay_X_8Dlan_319
321. NUCLEO-F411RE_PCB_TOP_Designators_Varsay_X_8Dlan_320
322. NUCLEO-F411RE_PCB_TOP_Designators_Varsay_X_8Dlan_321
323. NUCLEO-F411RE_PCB_TOP_Designators_Varsay_X_8Dlan_322
324. NUCLEO-F411RE_PCB_TOP_Designators_Varsay_X_8Dlan_323
325. NUCLEO-F411RE_PCB_TOP_Designators_Varsay_X_8Dlan_324
326. NUCLEO-F411RE_PCB_TOP_Designators_Varsay_X_8Dlan_325
327. NUCLEO-F411RE_PCB_TOP_Designators_Varsay_X_8Dlan_326
328. NUCLEO-F411RE_PCB_TOP_Designators_Varsay_X_8Dlan_327
329. NUCLEO-F411RE_PCB_TOP_Designators_Varsay_X_8Dlan_328
330. NUCLEO-F411RE_PCB_TOP_Designators_Varsay_X_8Dlan_329
331. NUCLEO-F411RE_PCB_TOP_Designators_Varsay_X_8Dlan_330
332. NUCLEO-F411RE_PCB_TOP_Designators_Varsay_X_8Dlan_331
333. NUCLEO-F411RE_PCB_TOP_Designators_Varsay_X_8Dlan_332
334. NUCLEO-F411RE_PCB_TOP_Designators_Varsay_X_8Dlan_333
335. NUCLEO-F411RE_PCB_TOP_Designators_Varsay_X_8Dlan_334
336. NUCLEO-F411RE_PCB_TOP_Designators_Varsay_X_8Dlan_335
337. NUCLEO-F411RE_PCB_TOP_Designators_Varsay_X_8Dlan_336
338. NUCLEO-F411RE_PCB_TOP_Designators_Varsay_X_8Dlan_337
339. NUCLEO-F411RE_PCB_TOP_Designators_Varsay_X_8Dlan_338
340. NUCLEO-F411RE_PCB_TOP_Designators_Varsay_X_8Dlan_339
341. NUCLEO-F411RE_PCB_TOP_Designators_Varsay_X_8Dlan_340
342. NUCLEO-F411RE_PCB_TOP_Designators_Varsay_X_8Dlan_341
343. NUCLEO-F411RE_PCB_TOP_Designators_Varsay_X_8Dlan_342
344. NUCLEO-F411RE_PCB_TOP_Designators_Varsay_X_8Dlan_343
345. NUCLEO-F411RE_PCB_TOP_Designators_Varsay_X_8Dlan_344
346. NUCLEO-F411RE_PCB_TOP_Designators_Varsay_X_8Dlan_345
347. NUCLEO-F411RE_PCB_TOP_Designators_Varsay_X_8Dlan_346
348. NUCLEO-F411RE_PCB_TOP_Designators_Varsay_X_8Dlan_347
349. NUCLEO-F411RE_PCB_TOP_Designators_Varsay_X_8Dlan_348
350. NUCLEO-F411RE_PCB_TOP_Designators_Varsay_X_8Dlan_349
351. NUCLEO-F411RE_PCB_TOP_Designators_Varsay_X_8Dlan_350
352. NUCLEO-F411RE_PCB_TOP_Designators_Varsay_X_8Dlan_351
353. NUCLEO-F411RE_PCB_TOP_Designators_Varsay_X_8Dlan_352
354. NUCLEO-F411RE_PCB_TOP_Designators_Varsay_X_8Dlan_353
355. NUCLEO-F411RE_PCB_TOP_Designators_Varsay_X_8Dlan_354
356. NUCLEO-F411RE_PCB_TOP_Designators_Varsay_X_8Dlan_355
357. NUCLEO-F411RE_PCB_TOP_Designators_Varsay_X_8Dlan_356
358. NUCLEO-F411RE_PCB_TOP_Designators_Varsay_X_8Dlan_357
359. NUCLEO-F411RE_PCB_TOP_Designators_Varsay_X_8Dlan_358
360. NUCLEO-F411RE_PCB_TOP_Designators_Varsay_X_8Dlan_359
361. NUCLEO-F411RE_PCB_TOP_Designators_Varsay_X_8Dlan_360
362. NUCLEO-F411RE_PCB_TOP_Designators_Varsay_X_8Dlan_361
363. NUCLEO-F411RE_PCB_TOP_Designators_Varsay_X_8Dlan_362
364. NUCLEO-F411RE_PCB_TOP_Designators_Varsay_X_8Dlan_363
365. NUCLEO-F411RE_PCB_TOP_Designators_Varsay_X_8Dlan_364
366. NUCLEO-F411RE_PCB_TOP_Designators_Varsay_X_8Dlan_365
367. NUCLEO-F411RE_PCB_TOP_Designators_Varsay_X_8Dlan_366
368. NUCLEO-F411RE_PCB_TOP_Designators_Varsay_X_8Dlan_367
369. NUCLEO-F411RE_PCB_TOP_Designators_Varsay_X_8Dlan_368
370. NUCLEO-F411RE_PCB_TOP_Designators_Varsay_X_8Dlan_369
371. NUCLEO-F411RE_PCB_TOP_Designators_Varsay_X_8Dlan_370
372. NUCLEO-F411RE_PCB_TOP_Designators_Varsay_X_8Dlan_371
373. NUCLEO-F411RE_PCB_TOP_Designators_Varsay_X_8Dlan_372
374. NUCLEO-F411RE_PCB_TOP_Designators_Varsay_X_8Dlan_373
375. NUCLEO-F411RE_PCB_TOP_Designators_Varsay_X_8Dlan_374
376. NUCLEO-F411RE_PCB_TOP_Designators_Varsay_X_8Dlan_375
377. NUCLEO-F411RE_PCB_TOP_Designators_Varsay_X_8Dlan_376
378. NUCLEO-F411RE_PCB_TOP_Designators_Varsay_X_8Dlan_377
379. NUCLEO-F411RE_PCB_TOP_Designators_Varsay_X_8Dlan_378
380. NUCLEO-F411RE_PCB_TOP_Designators_Varsay_X_8Dlan_379
381. NUCLEO-F411RE_PCB_TOP_Designators_Varsay_X_8Dlan_380
382. NUCLEO-F411RE_PCB_TOP_Designators_Varsay_X_8Dlan_381
383. NUCLEO-F411RE_PCB_TOP_Designators_Varsay_X_8Dlan_382
384. NUCLEO-F411RE_PCB_TOP_Designators_Varsay_X_8Dlan_383
385. NUCLEO-F411RE_PCB_TOP_Designators_Varsay_X_8Dlan_384
386. NUCLEO-F411RE_PCB_TOP_Designators_Varsay_X_8Dlan_385
387. NUCLEO-F411RE_PCB_TOP_Designators_Varsay_X_8Dlan_386
388. NUCLEO-F411RE_PCB_TOP_Designators_Varsay_X_8Dlan_387
389. NUCLEO-F411RE_PCB_TOP_Designators_Varsay_X_8Dlan_388
390. NUCLEO-F411RE_PCB_TOP_Designators_Varsay_X_8Dlan_389
391. NUCLEO-F411RE_PCB_TOP_Designators_Varsay_X_8Dlan_390
392. NUCLEO-F411RE_PCB_TOP_Designators_Varsay_X_8Dlan_391
393. NUCLEO-F411RE_PCB_TOP_Designators_Varsay_X_8Dlan_392
394. NUCLEO-F411RE_PCB_TOP_Designators_Varsay_X_8Dlan_393
395. NUCLEO-F411RE_PCB_TOP_Designators_Varsay_X_8Dlan_394
396. NUCLEO-F411RE_PCB_TOP_Designators_Varsay_X_8Dlan_395
397. NUCLEO-F411RE_PCB_TOP_Designators_Varsay_X_8Dlan_396
398. NUCLEO-F411RE_PCB_TOP_Designators_Varsay_X_8Dlan_397
399. NUCLEO-F411RE_PCB_TOP_Designators_Varsay_X_8Dlan_398
400. NUCLEO-F411RE_PCB_TOP_Designators_Varsay_X_8Dlan_399
401. NUCLEO-F411RE_PCB_TOP_Designators_Varsay_X_8Dlan_400
402. NUCLEO-F411RE_PCB_TOP_Designators_Varsay_X_8Dlan_401
403. NUCLEO-F411RE_PCB_TOP_Designators_Varsay_X_8Dlan_402
404. NUCLEO-F411RE_PCB_TOP_Designators_Varsay_X_8Dlan_403
405. NUCLEO-F411RE_PCB_TOP_Designators_Varsay_X_8Dlan_404
406. NUCLEO-F411RE_PCB_TOP_Designators_Varsay_X_8Dlan_405
407. NUCLEO-F411RE_PCB_TOP_Designators_Varsay_X_8Dlan_406
408. NUCLEO-F411RE_PCB_TOP_Designators_Varsay_X_8Dlan_407
409. NUCLEO-F411RE_PCB_TOP_Designators_Varsay_X_8Dlan_408
410. NUCLEO-F411RE_PCB_TOP_Designators_Varsay_X_8Dlan_409
411. NUCLEO-F411RE_PCB_TOP_Designators_Varsay_X_8Dlan_410
412. NUCLEO-F411RE_PCB_TOP_Designators_Varsay_X_8Dlan_411
413. NUCLEO-F411RE_PCB_TOP_Designators_Varsay_X_8Dlan_412
414. NUCLEO-F411RE_PCB_TOP_Designators_Varsay_X_8Dlan_413
415. NUCLEO-F411RE_PCB_TOP_Designators_Varsay_X_8Dlan_414
416. NUCLEO-F411RE_PCB_TOP_Designators_Varsay_X_8Dlan_415
417. NUCLEO-F411RE_PCB_TOP_Designators_Varsay_X_8Dlan_416
418. NUCLEO-F411RE_PCB_TOP_Designators_Varsay_X_8Dlan_417
419. NUCLEO-F411RE_PCB_TOP_Designators_Varsay_X_8Dlan_418
420. NUCLEO-F411RE_PCB_TOP_Designators_Varsay_X_8Dlan_419
421. NUCLEO-F411RE_PCB_TOP_Designators_Varsay_X_8Dlan_420
422. NUCLEO-F411RE_PCB_TOP_Designators_Varsay_X_8Dlan_421
423. NUCLEO-F411RE_PCB_TOP_Designators_Varsay_X_8Dlan_422
424. NUCLEO-F411RE_PCB_TOP_Designators_Varsay_X_8Dlan_423
425. NUCLEO-F411RE_PCB_TOP_Designators_Varsay_X_8Dlan_424
426. NUCLEO-F411RE_PCB_TOP_Designators_Varsay_X_8Dlan_425
427. NUCLEO-F411RE_PCB_TOP_Designators_Varsay_X_8Dlan_426
428. NUCLEO-F411RE_PCB_TOP_Designators_Varsay_X_8Dlan_427
429. NUCLEO-F411RE_PCB_TOP_Designators_Varsay_X_8Dlan_428
430. NUCLEO-F411RE_PCB_TOP_Designators_Varsay_X_8Dlan_429
431. NUCLEO-F411RE_PCB_TOP_Designators_Varsay_X_8Dlan_430
432. NUCLEO-F411RE_PCB_TOP_Designators_Varsay_X_8Dlan_431
433. NUCLEO-F411RE_PCB_TOP_Designators_Varsay_X_8Dlan_432
434. NUCLEO-F411RE_PCB_TOP_Designators_Varsay_X_8Dlan_433
435. NUCLEO-F411RE_PCB_TOP_Designators_Varsay_X_8Dlan_434
436. NUCLEO-F411RE_PCB_TOP_Designators_Varsay_X_8Dlan_435
437. NUCLEO-F411RE_PCB_TOP_Designators_Varsay_X_8Dlan_436
438. NUCLEO-F411RE_PCB_TOP_Designators_Varsay_X_8Dlan_437
439. NUCLEO-F411RE_PCB_TOP_Designators_Varsay_X_8Dlan_438
440. NUCLEO-F411RE_PCB_TOP_Designators_Varsay_X_8Dlan_439
441. NUCLEO-F411RE_PCB_TOP_Designators_Varsay_X_8Dlan_440
442. NUCLEO-F411RE_PCB_TOP_Designators_Varsay_X_8Dlan_441
443. NUCLEO-F411RE_PCB_TOP_Designators_Varsay_X_8Dlan_442
444. NUCLEO-F411RE_PCB_TOP_Designators_Varsay_X_8Dlan_443
445. NUCLEO-F411RE_PCB_TOP_Designators_Varsay_X_8Dlan_444
446. NUCLEO-F411RE_PCB_TOP_Designators_Varsay_X_8Dlan_445
447. NUCLEO-F411RE_PCB_TOP_Designators_Varsay_X_8Dlan_446
448. NUCLEO-F411RE_PCB_TOP_Designators_Varsay_X_8Dlan_447
449. NUCLEO-F411RE_PCB_TOP_Designators_Varsay_X_8Dlan_448
450. NUCLEO-F411RE_PCB_TOP_Designators_Varsay_X_8Dlan_449
451. NUCLEO-F411RE_PCB_TOP_Designators_Varsay_X_8Dlan_450
452. NUCLEO-F411RE_PCB_TOP_Designators_Varsay_X_8Dlan_451
453. NUCLEO-F411RE_PCB_TOP_Designators_Varsay_X_8Dlan_452
454. NUCLEO-F411RE_PCB_TOP_Designators_Varsay_X_8Dlan_453
455. NUCLEO-F411RE_PCB_TOP_Designators_Varsay_X_8Dlan_454
456. NUCLEO-F411RE_PCB_TOP_Designators_Varsay_X_8Dlan_455
457. NUCLEO-F411RE_PCB_TOP_Designators_Varsay_X_8Dlan_456
458. NUCLEO-F411RE_PCB_TOP_Designators_Varsay_X_8Dlan_457
459. NUCLEO-F411RE_PCB_TOP_Designators_Varsay_X_8Dlan_458
460. NUCLEO-F411RE_PCB_TOP_Designators_Varsay_X_8Dlan_459
461. NUCLEO-F411RE_PCB_TOP_Designators_Varsay_X_8Dlan_460
462. NUCLEO-F411RE_PCB_TOP_Designators_Varsay_X_8Dlan_461
463. NUCLEO-F411RE_PCB_TOP_Designators_Varsay_X_8Dlan_462
464. NUCLEO-F411RE_PCB_TOP_Designators_Varsay_X_8Dlan_463
465. NUCLEO-F411RE_PCB_TOP_Designators_Varsay_X_8Dlan_464
466. NUCLEO-F411RE_PCB_TOP_Designators_Varsay_X_8Dlan_465
467. NUCLEO-F411RE_PCB_TOP_Designators_Varsay_X_8Dlan_466
468. NUCLEO-F411RE_PCB_TOP_Designators_Varsay_X_8Dlan_467
469. NUCLEO-F411RE_PCB_TOP_Designators_Varsay_X_8Dlan_468
470. NUCLEO-F411RE_PCB_TOP_Designators_Varsay_X_8Dlan_469
471. NUCLEO-F411RE_PCB_TOP_Designators_Varsay_X_8Dlan_470
472. NUCLEO-F411RE_PCB_TOP_Designators_Varsay_X_8Dlan_471
473. NUCLEO-F411RE_PCB_TOP_Designators_Varsay_X_8Dlan_472
474. NUCLEO-F411RE_PCB_TOP_Designators_Varsay_X_8Dlan_473
475. NUCLEO-F411RE_PCB_TOP_Designators_Varsay_X_8Dlan_474
476. NUCLEO-F411RE_PCB_TOP_Designators_Varsay_X_8Dlan_475
477. NUCLEO-F411RE_PCB_TOP_Designators_Varsay_X_8Dlan_476
478. NUCLEO-F411RE_PCB_TOP_Designators_Varsay_X_8Dlan_477
479. NUCLEO-F411RE_PCB_TOP_Designators_Varsay_X_8Dlan_478
480. NUCLEO-F411RE_PCB_TOP_Designators_Varsay_X_8Dlan_479
481. NUCLEO-F411RE_PCB_TOP_Designators_Varsay_X_8Dlan_480
482. NUCLEO-F411RE_PCB_TOP_Designators_Varsay_X_8Dlan_481
483. NUCLEO-F411RE_PCB_TOP_Designators_Varsay_X_8Dlan_482
484. NUCLEO-F411RE_PCB_TOP_Designators_Varsay_X_8Dlan_483
485. NUCLEO-F411RE_PCB_TOP_Designators_Varsay_X_8Dlan_484
486. NUCLEO-F411RE_PCB_TOP_Designators_Varsay_X_8Dlan_485
487. NUCLEO-F411RE_PCB_TOP_Designators_Varsay_X_8Dlan_486
488. NUCLEO-F411RE_PCB_TOP_Designators_Varsay_X_8Dlan_487
489. NUCLEO-F411RE_PCB_TOP_Designators_Varsay_X_8Dlan_488
490. NUCLEO-F411RE_PCB_TOP_Designators_Varsay_X_8Dlan_489
491. NUCLEO-F411RE_PCB_TOP_Designators_Varsay_X_8Dlan_490
492. NUCLEO-F411RE_PCB_TOP_Designators_Varsay_X_8Dlan_491
493. NUCLEO-F411RE_PCB_TOP_Designators_Varsay_X_8Dlan_492
494. NUCLEO-F411RE_PCB_TOP_Designators_Varsay_X_8Dlan_493
495. NUCLEO-F411RE_PCB_TOP_Designators_Varsay_X_8Dlan_494
496. NUCLEO-F411RE_PCB_TOP_Designators_Varsay_X_8Dlan_495
497. NUCLEO-F411RE_PCB_TOP_Designators_Varsay_X_8Dlan_496
498. NUCLEO-F411RE_PCB_TOP_Designators_Varsay_X_8Dlan_497
499. NUCLEO-F411RE_PCB_TOP_Designators_Varsay_X_8Dlan_498
500. NUCLEO-F411RE_PCB_TOP_Designators_Varsay_X_8Dlan_499
501. NUCLEO-F411RE_PCB_TOP_Designators_Varsay_X_8Dlan_500
502. NUCLEO-F411RE_PCB_TOP_Designators_Varsay_X_8Dlan_501
503. NUCLEO-F411RE_PCB_TOP_Designators_Varsay_X_8Dlan_502
504. NUCLEO-F411RE_PCB_TOP_Designators_Varsay_X_8Dlan_503
505. NUCLEO-F411RE_PCB_TOP_Designators_Varsay_X_8Dlan_504
506. NUCLEO-F411RE_PCB_TOP_Designators_Varsay_X_8Dlan_505
507. NUCLEO-F411RE_PCB_TOP_Designators_Varsay_X_8Dlan_506
508. NUCLEO-F411RE_PCB_TOP_Designators_Varsay_X_8Dlan_507
509. NUCLEO-F411RE_PCB_TOP_Designators_Varsay_X_8Dlan_508
510. NUCLEO-F411RE_PCB_TOP_Designators_Varsay_X_8Dlan_509
511. NUCLEO-F411RE_PCB_TOP_Designators_Varsay_X_8Dlan_510
512. NUCLEO-F411RE_PCB_TOP_Designators_Varsay_X_8Dlan_511
513. NUCLEO-F411RE_PCB_TOP_Designators_Varsay_X_8Dlan_512
514. NUCLEO-F411RE_PCB_TOP_Designators_Varsay_X_8Dlan_513
515. NUCLEO-F411RE_PCB_TOP_Designators_Varsay_X_8Dlan_514
516. NUCLEO-F411RE_PCB_TOP_Designators_Varsay_X_8Dlan_515
517. NUCLEO-F411RE_PCB_TOP_Designators_Varsay_X_8Dlan_516
518. NUCLEO-F411RE_PCB_TOP_Designators_Varsay_X_8Dlan_517
519. NUCLEO-F411RE_PCB_TOP_Designators_Varsay_X_8Dlan_518
520. NUCLEO-F411RE_PCB_TOP_Designators_Varsay_X_8Dlan_519
521. NUCLEO-F411RE_PCB_TOP_Designators_Varsay_X_8Dlan_520
522. NUCLEO-F411RE_PCB_TOP_Designators_Varsay_X_8Dlan_521
523. NUCLEO-F411RE_PCB_TOP_Designators_Varsay_X_8Dlan_522
524. NUCLEO-F411RE_PCB_TOP_Designators_Varsay_X_8Dlan_523
525. NUCLEO-F411RE_PCB_TOP_Designators_Varsay_X_8Dlan_524
526. NUCLEO-F411RE_PCB_TOP_Designators_Varsay_X_8Dlan_525
527. NUCLEO-F411RE_PCB_TOP_Designators_Varsay_X_8Dlan_526
528. NUCLEO-F411RE_PCB_TOP_Designators_Varsay_X_8Dlan_527
529. NUCLEO-F411RE_PCB_TOP_Designators_Varsay_X_8Dlan_528
530. NUCLEO-F411RE_PCB_TOP_Designators_Varsay_X_8Dlan_529
531. NUCLEO-F411RE_PCB_TOP_Designators_Varsay_X_8Dlan_530
532. NUCLEO-F411RE_PCB_TOP_Designators_Varsay_X_8Dlan_531
